# Autodesk Inventor assembly: Gantry_y
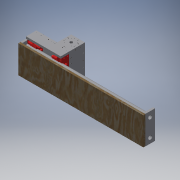
[picture p0: Inventor's stored thumbnail of the model, 180x180]
Saved by Autodesk Inventor 2016 SP2 (Build 200236200, 236)
## iProperties
Created: 2017-09-10
Part Number: Gantry_y
Document SubType Name: Assembly
Designer: Admin
Mass: 5647.73 g
Surface Area: 13929.1 cm^2
Volume: 6433.97 cm^3
Density: 0.877798 g/cm^3
Author: Admin
## Documents named in this file (5)
- E:\DATA\Inventor\AtongJali_v2\Gantry_y.iam
- E:\DATA\Inventor\AtongJali_v2\sideskirt_mount_lower.iam
- E:\DATA\Inventor\AtongJali_v2\batang_900.ipt
- E:\DATA\Inventor\AtongJali_v2\Base_wood.ipt
- E:\DATA\Inventor\AtongJali_v2\gantry_y_holder.ipt
## Components (6 placed, 4 different names)
1. sideskirt_mount_lower:1 [sub-assembly] — Cylindrical:1, Cylindrical:2, Mate:1
2. batang_900:1 — Cylindrical:2, Rotational:2, Rotational:4
3. batang_900:2 — Cylindrical:1, Rotational:1, Rotational:3
4. Base_wood:1 — Rigid:1
5. gantry_y_holder:1 — Rotational:1, Rotational:2, Rigid:1
6. gantry_y_holder:2 — Rotational:3, Rotational:4, Mate:1
## Relationships (8: RevoluteJoint 4, CylindricalJoint 2, WeldJoint 1, Mate 1)
- Cylindrical:1: sideskirt_mount_lower:1 ↔ batang_900:2
- Cylindrical:2: sideskirt_mount_lower:1 ↔ batang_900:1
- Rotational:1 [RevoluteJoint]: batang_900:2 ↔ gantry_y_holder:1
- Rotational:2 [RevoluteJoint]: batang_900:1 ↔ gantry_y_holder:1
- Rotational:3 [RevoluteJoint]: batang_900:2 ↔ gantry_y_holder:2
- Rotational:4 [RevoluteJoint]: batang_900:1 ↔ gantry_y_holder:2
- Rigid:1 [WeldJoint]: Base_wood:1 ↔ gantry_y_holder:1
- Mate:1 (620 mm): sideskirt_mount_lower:1 ↔ gantry_y_holder:2
